# Autodesk Inventor assembly: Roller
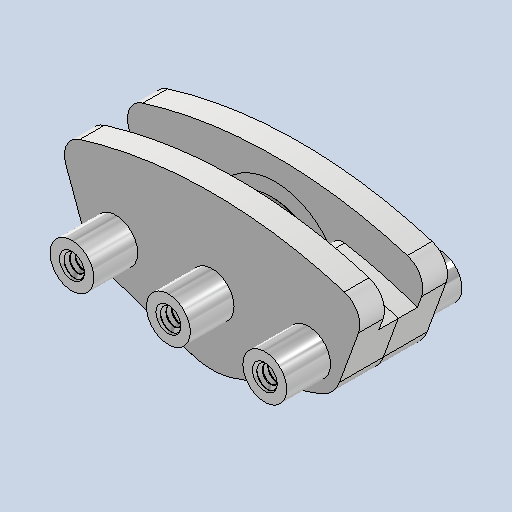
[picture p0: Inventor's stored thumbnail of the model, 512x512]
Saved by Autodesk Inventor 2023.2 (Build 272271000, 271)
## iProperties
Created: 2023-06-11
Part Number: Roller
Document SubType Name: Assembly
Designer: Nathan Cai
Mass: 16.0173 g
Surface Area: 88.1517 cm^2
Volume: 7.85874 cm^3
Density: 2.03816 g/cm^3
Author: Nathan Cai
## Documents named in this file (4)
- E:\Documents\Inventor\Law - V1.0\Roller.iam
- E:\Documents\Inventor\Law - V1.0\Ring Bushing.ipt
- E:\Documents\Inventor\Law - V1.0\5-8in OD Ball Bearing.ipt
- E:\Documents\Inventor\Law - V1.0\Standoff 1in.ipt
## Components (6 placed, 3 different names)
1. Ring Bushing:1 — Mate:1, Mate:2, Mate:3, Mate:6, Mate:7, Mate:9, Flush:2
2. Ring Bushing:2 — Mate:2, Mate:3, Mate:8, Mate:9
3. 5-8in OD Ball Bearing:1 — Mate:1, Mate:8, Mate:10
4. Standoff 1in:1 — Mate:6, Flush:1, Flush:2, Flush:3
5. Standoff 1in:2 — Mate:7, Flush:1
6. Standoff 1in:3 — Mate:10, Flush:3
## Relationships (11: Mate 8, Flush 3)
- Mate:1: Ring Bushing:1 ↔ 5-8in OD Ball Bearing:1
- Mate:2: Ring Bushing:1 ↔ Ring Bushing:2
- Mate:3: Ring Bushing:1 ↔ Ring Bushing:2
- Mate:6: Ring Bushing:1 ↔ Standoff 1in:1
- Mate:7: Ring Bushing:1 ↔ Standoff 1in:2
- Flush:1: Standoff 1in:1 ↔ Standoff 1in:2
- Mate:8: Ring Bushing:2 ↔ 5-8in OD Ball Bearing:1
- Mate:9: Ring Bushing:1 ↔ Ring Bushing:2
- Flush:2 (-6.35 mm): Ring Bushing:1 ↔ Standoff 1in:1
- Mate:10: 5-8in OD Ball Bearing:1 ↔ Standoff 1in:3
- Flush:3: Standoff 1in:1 ↔ Standoff 1in:3
